# Autodesk Inventor assembly: Assembly_NV__Optical_Modules
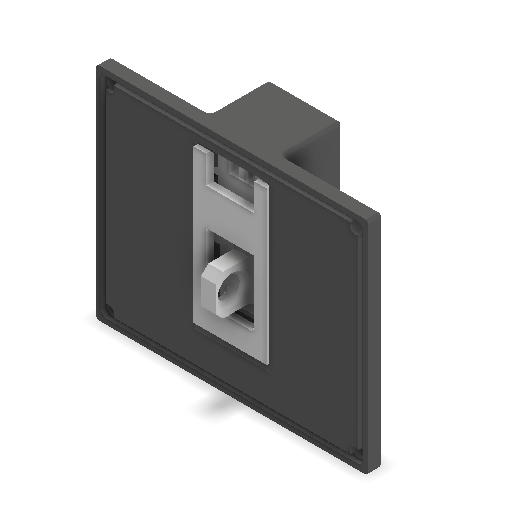
[picture p0: Inventor's stored thumbnail of the model, 512x512]
Saved by Autodesk Inventor 2026.1 (Build 301233020, 233B)
## iProperties
Created: 2026-02-05
Part Number: Assembly_NV__Optical_Modules
Document SubType Name: Assembly
Designer: samuel
Author: samuel
## Documents named in this file (9)
- E:\Fraunhofer\Design\Assembly_NV__Optical_Modules.iam
- E:\Fraunhofer\Design\Box_lid_v4.ipt
- E:\Fraunhofer\Design\Assembly_Optical_Module.iam
- E:\Fraunhofer\Design\Assembly_NV_Module.iam
- E:\Fraunhofer\Design\Modules_cover.ipt
- E:\Fraunhofer\Design\Parts\dupont-jumper-wire-1.snapshot.3\Dupont Jumper Wire F-F\Dupont Jumper Wire F-F\Dupont Jumper Wire F-F - black.ipt
- E:\Fraunhofer\Design\Parts\dupont-jumper-wire-1.snapshot.3\Dupont Jumper Wire F-F\Dupont Jumper Wire F-F\Dupont Jumper Wire F-F - green.ipt
- E:\Fraunhofer\Design\Parts\dupont-jumper-wire-1.snapshot.3\Dupont Jumper Wire F-F\Dupont Jumper Wire F-F\Dupont Jumper Wire F-F - yellow.ipt
- E:\Fraunhofer\Design\Parts\dupont-jumper-wire-1.snapshot.3\Dupont Jumper Wire F-F\Dupont Jumper Wire F-F\Dupont Jumper Wire F-F.ipt
## Components (8 placed, 8 different names)
1. Box_lid_v4:1 — Mate:2, Mate:3, Mate:4, Mate:5, Mate:7, Mate:8
2. Assembly_Optical_Module:1 [sub-assembly] — Mate:2, Mate:3, Flush:1, Mate:12, Flush:7, Mate:14
3. Assembly_NV_Module:1 [sub-assembly] — Mate:4, Mate:5, Flush:1, Mate:11, Flush:4, Mate:13
4. Modules_cover:1 — Mate:7, Mate:8
5. Dupont Jumper Wire F-F - black:1 — Mate:10, Flush:5, Flush:6
6. Dupont Jumper Wire F-F - green:1 — Mate:9, Flush:2, Flush:3
7. Dupont Jumper Wire F-F - yellow:1 — Mate:9, Flush:2, Flush:3, Mate:11, Flush:4, Mate:13
8. Dupont Jumper Wire F-F:1 — Mate:10, Flush:5, Flush:6, Mate:12, Flush:7, Mate:14
## Relationships (19: Mate 12, Flush 7)
- Mate:2: Box_lid_v4:1 ↔ Assembly_Optical_Module:1
- Mate:3: Box_lid_v4:1 ↔ Assembly_Optical_Module:1
- Mate:4: Box_lid_v4:1 ↔ Assembly_NV_Module:1
- Mate:5: Box_lid_v4:1 ↔ Assembly_NV_Module:1
- Flush:1: Assembly_Optical_Module:1 ↔ Assembly_NV_Module:1
- Mate:7: Box_lid_v4:1 ↔ Modules_cover:1
- Mate:8: Box_lid_v4:1 ↔ Modules_cover:1
- Mate:9 (3 mm): Dupont Jumper Wire F-F - green:1 ↔ Dupont Jumper Wire F-F - yellow:1
- Mate:10 (3 mm): Dupont Jumper Wire F-F - black:1 ↔ Dupont Jumper Wire F-F:1
- Flush:2: Dupont Jumper Wire F-F - green:1 ↔ Dupont Jumper Wire F-F - yellow:1
- Flush:3: Dupont Jumper Wire F-F - green:1 ↔ Dupont Jumper Wire F-F - yellow:1
- Mate:11: Assembly_NV_Module:1 ↔ Dupont Jumper Wire F-F - yellow:1
- Flush:4: Assembly_NV_Module:1 ↔ Dupont Jumper Wire F-F - yellow:1
- Flush:5: Dupont Jumper Wire F-F - black:1 ↔ Dupont Jumper Wire F-F:1
- Flush:6: Dupont Jumper Wire F-F - black:1 ↔ Dupont Jumper Wire F-F:1
- Mate:12: Assembly_Optical_Module:1 ↔ Dupont Jumper Wire F-F:1
- Flush:7: Assembly_Optical_Module:1 ↔ Dupont Jumper Wire F-F:1
- Mate:13 (0.5 mm): Assembly_NV_Module:1 ↔ Dupont Jumper Wire F-F - yellow:1
- Mate:14 (1 mm): Assembly_Optical_Module:1 ↔ Dupont Jumper Wire F-F:1
